# Autodesk Inventor assembly: Wasabi
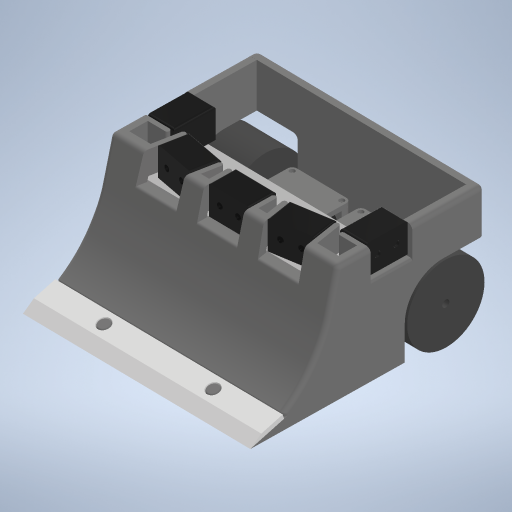
[picture p0: Inventor's stored thumbnail of the model, 512x512]
Saved by Autodesk Inventor 2024 (Build 280153000, 153)
## iProperties
Created: 2023-10-20
Part Number: Wasabi
Document SubType Name: Assembly
Designer: kdcao
Author: kdcao
## Documents named in this file (9)
- C:\Users\kdcao\Documents\GitHub\wasabi2\Wasabi\Wasabi.iam
- C:\Users\kdcao\Documents\GitHub\wasabi2\Wasabi\Body\Body.ipt
- C:\Users\kdcao\Documents\GitHub\wasabi2\Wasabi\Parts\battery.ipt
- C:\Users\kdcao\Documents\GitHub\wasabi2\Wasabi\Parts\qtr-1a-reflectance-sensor.ipt
- C:\Users\kdcao\Documents\GitHub\wasabi2\Wasabi\Parts\wheel.ipt
- C:\Users\kdcao\Documents\GitHub\wasabi2\Wasabi\Parts\micro-metal-gearmotor-standard.ipt
- C:\Users\kdcao\Documents\GitHub\wasabi2\Wasabi\Parts\IR sensor.ipt
- C:\Users\kdcao\Documents\GitHub\wasabi2\Wasabi\Parts\Blade.ipt
- C:\Users\kdcao\Documents\GitHub\wasabi2\Wasabi\Parts\IR sensor_MIR1.ipt
## Components (14 placed, 8 different names)
1. Body:1 — Angle:1, Flush:3, Mate:3, Flush:4, Tangent:1, Tangent:2, Flush:5, Mate:5, Flush:6, Tangent:3, Tangent:4, Flush:7, Angle:2, Mate:13, Angle:3, Mate:15, Mate:17, Mate:18, Rigid:2, Rigid:3, Rigid:4, Flush:8, Mate:20
2. battery:1 — Angle:1, Flush:3, Mate:3, Flush:4, Mate:9, Mate:11, Mate:12, Mate:19
3. qtr-1a-reflectance-sensor:1 — Rigid:3
4. qtr-1a-reflectance-sensor:2 — Rigid:2
5. wheel:2 — Tangent:1, Tangent:2, Flush:5, Cylindrical:1, Mate:4
6. micro-metal-gearmotor-standard:2 — Cylindrical:1, Mate:4
7. wheel:3 — Rotational:1, Flush:6, Tangent:3, Tangent:4
8. micro-metal-gearmotor-standard:3 — Mate:5, Rotational:1
9. IR sensor:1 — Mate:9, Flush:7, Mate:16
10. IR sensor:2 — Mate:11, Angle:2, Mate:13, Mate:18
11. IR sensor:3 — Mate:12, Angle:3, Mate:15, Mate:16, Mate:17
12. IR sensor:4 — Mate:19, Flush:8, Mate:20
13. Blade:1 — Rigid:4
14. IR sensor_MIR1:1
## Relationships (31: Mate 13, Flush 6, Tangent 4, Angle 3, WeldJoint 3, CylindricalJoint 1, RevoluteJoint 1)
- Angle:1 (0 deg): Body:1 ↔ battery:1
- Flush:3: Body:1 ↔ battery:1
- Mate:3: Body:1 ↔ battery:1
- Flush:4: Body:1 ↔ battery:1
- Tangent:1 (1 mm): Body:1 ↔ wheel:2
- Tangent:2 (1 mm): Body:1 ↔ wheel:2
- Flush:5: Body:1 ↔ wheel:2
- Cylindrical:1: wheel:2 ↔ micro-metal-gearmotor-standard:2
- Mate:4: wheel:2 ↔ micro-metal-gearmotor-standard:2
- Mate:5: Body:1 ↔ micro-metal-gearmotor-standard:3
- Rotational:1 [RevoluteJoint]: wheel:3 ↔ micro-metal-gearmotor-standard:3
- Flush:6: Body:1 ↔ wheel:3
- Tangent:3 (1 mm): Body:1 ↔ wheel:3
- Tangent:4 (1 mm): Body:1 ↔ wheel:3
- Mate:9: battery:1 ↔ IR sensor:1
- Flush:7: Body:1 ↔ IR sensor:1
- Mate:11: battery:1 ↔ IR sensor:2
- Mate:12: battery:1 ↔ IR sensor:3
- Angle:2 (10 deg): Body:1 ↔ IR sensor:2
- Mate:13 (-15 mm): Body:1 ↔ IR sensor:2
- Angle:3 (-10 deg): Body:1 ↔ IR sensor:3
- Mate:15 (15 mm): Body:1 ↔ IR sensor:3
- Mate:16: IR sensor:1 ↔ IR sensor:3
- Mate:17: Body:1 ↔ IR sensor:3
- Mate:18: Body:1 ↔ IR sensor:2
- Rigid:2 [WeldJoint]: Body:1 ↔ qtr-1a-reflectance-sensor:2
- Rigid:3 [WeldJoint]: Body:1 ↔ qtr-1a-reflectance-sensor:1
- Rigid:4 [WeldJoint]: Body:1 ↔ Blade:1
- Mate:19: battery:1 ↔ IR sensor:4
- Flush:8 (-2 mm): Body:1 ↔ IR sensor:4
- Mate:20: Body:1 ↔ IR sensor:4
